# Autodesk Inventor assembly: Working Encoder
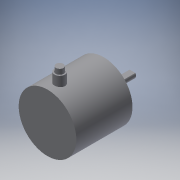
[picture p0: Inventor's stored thumbnail of the model, 180x180]
Saved by Autodesk Inventor 2016 (Build 200138000, 138)
## iProperties
Created: 2017-05-30
Part Number: Working Encoder
Document SubType Name: Assembly
Designer: M220404
Author: M220404
## Documents named in this file (3)
- C:\Users\M220404\Desktop\Working Encoder.iam
- C:\Users\M220404\Desktop\Belt Encoder Body.ipt
- C:\Users\M220404\Desktop\Belt encoder shaft.ipt
## Components (2 placed, 2 different names)
1. Belt Encoder Body:1 — Mate:1, Mate:2
2. Belt encoder shaft:1 — Mate:1, Mate:2
## Relationships (2: Mate 2)
- Mate:1: Belt Encoder Body:1 ↔ Belt encoder shaft:1
- Mate:2: Belt Encoder Body:1 ↔ Belt encoder shaft:1
